# Autodesk Inventor assembly: 2016-02-07-RhinoRobotV13
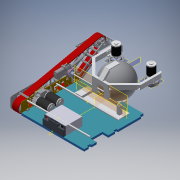
[picture p0: Inventor's stored thumbnail of the model, 180x180]
Saved by Autodesk Inventor 2016 SP1 (Build 200210100, 210)
## iProperties
Created: 2016-01-23
Part Number: 2016-02-07-RhinoRobotV13
Document SubType Name: Assembly
Designer: steele
Mass: 23360.3 g
Surface Area: 43274.3 cm^2
Volume: 23034.6 cm^3
Density: 1.01414 g/cm^3
Author: steele
## Documents named in this file (8)
- C:\snobotics\CAD-Development\robSteele\SnoBotics2016\2016-01-07-RhinoRobot\2016-02-07-RhinoRobotV13.iam
- C:\snobotics\CAD-Development\robSteele\SnoBotics2016\RhinoTrackDriveModule\am-3322+RhinoTrackDriveModule.iam
- C:\snobotics\CAD-Development\robSteele\SnoBotics2016\RhinoBottomFloorOptions\RhinoBottomFloorPlate01.ipt
- C:\snobotics\autodesk\2016\FRC KOP 2016\Electrical\fc16-036_Battery.iam
- C:\snobotics\CAD-Development\robSteele\SnoBotics2016\AM Parts\Churo_21_5_inches.ipt
- C:\snobotics\CAD-Development\robSteele\SnoBotics2016\AM Parts\am-3352 Rhino Front Left Bumper Bracket.ipt
- C:\snobotics\CAD-Development\robSteele\SnoBotics2016\AM Parts\am-0077a-500 Key Hub r2.ipt
- C:\snobotics\CAD-Development\robSteele\SnoBotics2016\2016-05-05-ShooterPrototype\ShooterAssemblyV05.iam
## Components (8 placed, 7 different names)
1. RhinoBottomFloorPlate01:1 — Mate:1, Flush:2, Flush:11, Flush:19, Flush:21, Mate:4, Flush:22
2. am-3322+RhinoTrackDriveModule:1 [sub-assembly] — Mate:1, Flush:2, Flush:11, Insert:1, Insert:6, Mate:2, Insert:8
3. Churo_21_5_inches:1 — Insert:1, Flush:18
4. Churo_21_5_inches:3 — Insert:6
5. fc16-036_Battery:1 [sub-assembly] — Mate:2, Flush:19
6. ShooterAssemblyV05:1 [sub-assembly] — Flush:21, Mate:3, Insert:9, Mate:4, Flush:22
7. am-3352 Rhino Front Left Bumper Bracket:1 — Insert:8
8. am-0077a-500 Key Hub r2:1 — Insert:9
## Relationships (14: Flush 6, Mate 4, Insert 4)
- Mate:1: RhinoBottomFloorPlate01:1 ↔ am-3322+RhinoTrackDriveModule:1
- Flush:2: RhinoBottomFloorPlate01:1 ↔ am-3322+RhinoTrackDriveModule:1
- Flush:11: RhinoBottomFloorPlate01:1 ↔ am-3322+RhinoTrackDriveModule:1
- Insert:1: am-3322+RhinoTrackDriveModule:1 ↔ Churo_21_5_inches:1
- Insert:6: am-3322+RhinoTrackDriveModule:1 ↔ Churo_21_5_inches:3
- Flush:18: Churo_21_5_inches:1
- Mate:2 (184.15 mm): am-3322+RhinoTrackDriveModule:1 ↔ fc16-036_Battery:1
- Flush:19: RhinoBottomFloorPlate01:1 ↔ fc16-036_Battery:1
- Flush:21: RhinoBottomFloorPlate01:1 ↔ ShooterAssemblyV05:1
- Mate:3: ShooterAssemblyV05:1
- Insert:8: am-3322+RhinoTrackDriveModule:1 ↔ am-3352 Rhino Front Left Bumper Bracket:1
- Insert:9: ShooterAssemblyV05:1 ↔ am-0077a-500 Key Hub r2:1
- Mate:4: RhinoBottomFloorPlate01:1 ↔ ShooterAssemblyV05:1
- Flush:22 (-63.5 mm): RhinoBottomFloorPlate01:1 ↔ ShooterAssemblyV05:1
## Named parameters: robotWidth = 660.4 mm, halfRobotWidth = 330.2 mm, maxPerimeter = 3048 mm, maxLength = 863.6 mm, widthOfTrack = 95.25 mm, boardWidth = 469.9 mm
